# Autodesk Inventor assembly: cnc vertex vasi
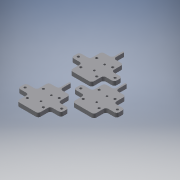
[picture p0: Inventor's stored thumbnail of the model, 180x180]
Saved by Autodesk Inventor 2016 SP1 (Build 200210100, 210)
## iProperties
Created: 2016-04-27
Part Number: cnc vertex vasi
Document SubType Name: Assembly
Designer: ubik
Author: ubik
## Documents named in this file (2)
- E:\GitHub\kossel-XXL\cnc vertex vasi.iam
- E:\GitHub\kossel-XXL\vertical carriage vasi.ipt
## Components (3 placed, 1 different names)
1. vertical carriage vasi:1 — Flush:1, Flush:2, Mate:1, Flush:3, Flush:4
2. vertical carriage vasi:2 — Flush:1, Mate:1, Flush:3, Mate:2
3. vertical carriage vasi:3 — Flush:2, Mate:2, Flush:4
## Relationships (6: Flush 4, Mate 2)
- Flush:1: vertical carriage vasi:1 ↔ vertical carriage vasi:2
- Flush:2: vertical carriage vasi:1 ↔ vertical carriage vasi:3
- Mate:1 (-90 mm): vertical carriage vasi:1 ↔ vertical carriage vasi:2
- Flush:3 (-34 mm): vertical carriage vasi:1 ↔ vertical carriage vasi:2
- Mate:2 (8 mm): vertical carriage vasi:2 ↔ vertical carriage vasi:3
- Flush:4: vertical carriage vasi:1 ↔ vertical carriage vasi:3
